# Autodesk Inventor assembly: Wind Tunnel Assembly 1
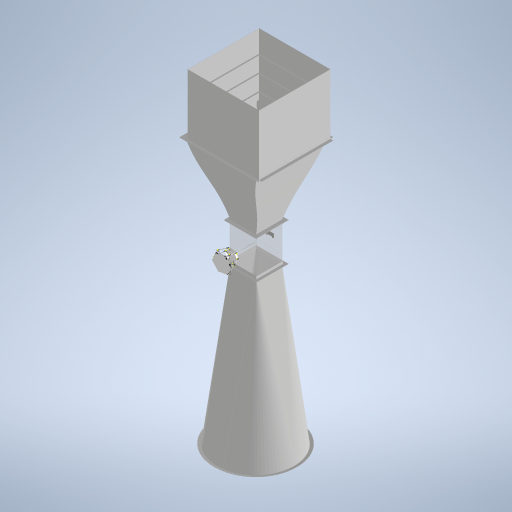
[picture p0: Inventor's stored thumbnail of the model, 512x512]
Saved by Autodesk Inventor 2023 (Build 270158000, 158)
## iProperties
Created: 2022-03-06
Part Number: Wind Tunnel Assembly 1
Document SubType Name: Assembly
Designer: calvi
Author: calvi
## Documents named in this file (6)
- C:\Users\earls\Documents\stewart-platform\CAD\Wind tunnel\Wind Tunnel Assembly 1.iam
- C:\Users\earls\Documents\stewart-platform\CAD\Wind tunnel\Entrance Assembly.iam
- C:\Users\earls\Documents\stewart-platform\CAD\Wind tunnel\Contraction Assembly.iam
- C:\Users\earls\Documents\stewart-platform\CAD\Wind tunnel\Diffuser.ipt
- C:\Users\earls\Documents\stewart-platform\CAD\Wind tunnel\updatedtestsectionassembly.iam
- C:\Users\earls\Documents\stewart-platform\CAD\St.iam
## Components (5 placed, 5 different names)
1. Entrance Assembly:1 [sub-assembly] — Flush:1, Flush:2, Mate:1
2. Contraction Assembly:1 [sub-assembly] — Flush:1, Flush:2, Mate:1, Flush:3, Mate:2, Flush:4
3. updatedtestsectionassembly:1 [sub-assembly] — Flush:3, Mate:2, Flush:4, Flush:5, Mate:3, Mate:4, Mate:5
4. Diffuser:1 — Flush:5, Mate:3
5. St:1 [sub-assembly] — Mate:4, Mate:5
## Relationships (10: Flush 5, Mate 5)
- Flush:1: Entrance Assembly:1 ↔ Contraction Assembly:1
- Flush:2: Entrance Assembly:1 ↔ Contraction Assembly:1
- Mate:1: Entrance Assembly:1 ↔ Contraction Assembly:1
- Flush:3: Contraction Assembly:1 ↔ updatedtestsectionassembly:1
- Mate:2: Contraction Assembly:1 ↔ updatedtestsectionassembly:1
- Flush:4: Contraction Assembly:1 ↔ updatedtestsectionassembly:1
- Flush:5: updatedtestsectionassembly:1 ↔ Diffuser:1
- Mate:3: updatedtestsectionassembly:1 ↔ Diffuser:1
- Mate:4: updatedtestsectionassembly:1 ↔ St:1
- Mate:5 (175 mm): updatedtestsectionassembly:1 ↔ St:1
